# Autodesk Inventor assembly: Handyhalterung_neu
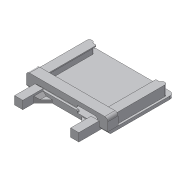
[picture p0: Inventor's stored thumbnail of the model, 180x180]
Saved by Autodesk Inventor 2013 (Build 170138000, 138)
## iProperties
Created: 2013-08-23
Part Number: Handyhalterung_neu
Document SubType Name: Assembly
Designer: Harald
Author: Harald
## Documents named in this file (6)
- C:\Users\Harald\Documents\Inventor\Handyhalterung\Handyhalterung_neu.iam
- C:\Users\Harald\Documents\Inventor\Handyhalterung\Grundplatte_zerlegt.ipt
- C:\Users\Harald\Documents\Inventor\Handyhalterung\Halter_links.ipt
- C:\Users\Harald\Documents\Inventor\Handyhalterung\Halter_rechts.ipt
- C:\Users\Harald\Documents\Inventor\Handyhalterung\USB-Halter.ipt
- C:\Users\Harald\Documents\Inventor\Handyhalterung\Galaxy S2.ipt
## Components (5 placed, 5 different names)
1. Grundplatte_zerlegt:1 — Passend:1, Passend:2, Winkel:1, Einfügen:1, Einfügen:2, Einfügen:3, Einfügen:4, Passend:4
2. Halter_links:1 — Passend:1, Passend:2, Winkel:1, Passend:3
3. Halter_rechts:1 — Einfügen:1, Einfügen:2
4. USB-Halter:1 — Einfügen:3, Einfügen:4, Passend:5
5. Galaxy S2:1 — Passend:3, Passend:4, Passend:5
## Relationships (10: Mate 5, Insert 4, Angle 1)
- Passend:1 [Mate]: Grundplatte_zerlegt:1 ↔ Halter_links:1
- Passend:2 [Mate]: Grundplatte_zerlegt:1 ↔ Halter_links:1
- Winkel:1 [Angle] (0 deg): Grundplatte_zerlegt:1 ↔ Halter_links:1
- Einfügen:1 [Insert]: Grundplatte_zerlegt:1 ↔ Halter_rechts:1
- Einfügen:2 [Insert]: Grundplatte_zerlegt:1 ↔ Halter_rechts:1
- Einfügen:3 [Insert]: Grundplatte_zerlegt:1 ↔ USB-Halter:1
- Einfügen:4 [Insert]: Grundplatte_zerlegt:1 ↔ USB-Halter:1
- Passend:3 [Mate]: Halter_links:1 ↔ Galaxy S2:1
- Passend:4 [Mate]: Grundplatte_zerlegt:1 ↔ Galaxy S2:1
- Passend:5 [Mate]: USB-Halter:1 ↔ Galaxy S2:1
